# Autodesk Inventor assembly: Assembly1DS
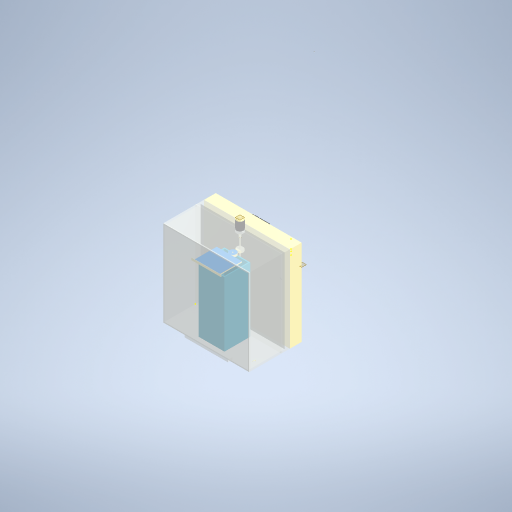
[picture p0: Inventor's stored thumbnail of the model, 512x512]
Saved by Autodesk Inventor 2024 (Build 280153000, 153)
## iProperties
Created: 2023-05-28
Part Number: Assembly1DS
Document SubType Name: Assembly
Designer: hithi
Author: hithi
## Documents named in this file (14)
- C:\Users\hithi\OneDrive\Documents\Assembly1DS.iam
- C:\Users\hithi\OneDrive\Documents\DS PART1.ipt
- C:\Users\hithi\OneDrive\Documents\BASE BOTTOM1.ipt
- C:\Users\hithi\OneDrive\Documents\DS PAERT 2 ALTER.ipt
- C:\Users\hithi\OneDrive\Desktop\Part16.ipt
- C:\Users\hithi\Downloads\16mhz crystal - measured\16mhz crystal - measured.ipt
- C:\Users\hithi\Downloads\arduino_MEGA2650\arduino_MEGA2650.iam
- C:\Users\hithi\Downloads\led\led.ipt
- C:\Users\hithi\Downloads\lmv358\lmv358.ipt
- C:\Users\hithi\Downloads\lp2985dgkr\lp2985dgkr.ipt
- C:\Users\hithi\Downloads\m7 diode\m7 diode.ipt
- C:\Users\hithi\Downloads\usb top contact\usb top contact.ipt
- C:\Users\hithi\Downloads\led-red-5mm-2.snapshot.1\BTG_901_BT_001_LED_5mm_Rot\LED_5mm_Rot.ipt
- C:\Users\hithi\Downloads\led-green-5mm-1.snapshot.1\BTG_901_BT_003_LED_5mm_Green\LED_5mm_Green.ipt
## Components (14 placed, 13 different names)
1. DS PART1:1 — Mate:1, Mate:2, Flush:1, Mate:4, Mate:5, Mate:6, Mate:7, Mate:8, Mate:9, Mate:10, Mate:11, Mate:12, Mate:14, Mate:15, Mate:16, Mate:17
2. BASE BOTTOM1:1 — Mate:1, Mate:3, Mate:5, Mate:6, Mate:7, Mate:8, Mate:13
3. BASE BOTTOM1:2 — Mate:9, Mate:10, Mate:11
4. DS PAERT 2 ALTER:1 — Mate:2, Flush:1, Mate:3, Mate:4
5. Part16:1 — Mate:12, Mate:13, Mate:14, Mate:15, Mate:16, Mate:17, Mate:18, Mate:19, Mate:20
6. arduino_MEGA2650:1 [sub-assembly] — Mate:18, Mate:19, Mate:20
7. led:1
8. lmv358:1
9. lp2985dgkr:1
10. m7 diode:1
11. usb top contact:2
12. 16mhz crystal - measured:6
13. LED_5mm_Rot:1
14. LED_5mm_Green:1
## Relationships (21: Mate 20, Flush 1)
- Mate:1: DS PART1:1 ↔ BASE BOTTOM1:1
- Mate:2: DS PART1:1 ↔ DS PAERT 2 ALTER:1
- Flush:1: DS PART1:1 ↔ DS PAERT 2 ALTER:1
- Mate:3: BASE BOTTOM1:1 ↔ DS PAERT 2 ALTER:1
- Mate:4: DS PART1:1 ↔ DS PAERT 2 ALTER:1
- Mate:5: DS PART1:1 ↔ BASE BOTTOM1:1
- Mate:6: DS PART1:1 ↔ BASE BOTTOM1:1
- Mate:7: DS PART1:1 ↔ BASE BOTTOM1:1
- Mate:8: DS PART1:1 ↔ BASE BOTTOM1:1
- Mate:9: DS PART1:1 ↔ BASE BOTTOM1:2
- Mate:10: DS PART1:1 ↔ BASE BOTTOM1:2
- Mate:11: DS PART1:1 ↔ BASE BOTTOM1:2
- Mate:12: DS PART1:1 ↔ Part16:1
- Mate:13: BASE BOTTOM1:1 ↔ Part16:1
- Mate:14: DS PART1:1 ↔ Part16:1
- Mate:15: DS PART1:1 ↔ Part16:1
- Mate:16: DS PART1:1 ↔ Part16:1
- Mate:17: DS PART1:1 ↔ Part16:1
- Mate:18: Part16:1 ↔ arduino_MEGA2650:1
- Mate:19: Part16:1 ↔ arduino_MEGA2650:1
- Mate:20 (7.62 mm): Part16:1 ↔ arduino_MEGA2650:1
